# Autodesk Inventor assembly: lemon shape asse
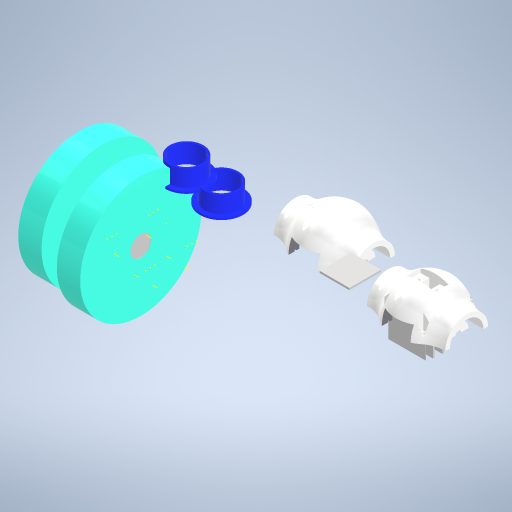
[picture p0: Inventor's stored thumbnail of the model, 512x512]
Saved by Autodesk Inventor 2023 (Build 270158000, 158)
## iProperties
Created: 2022-11-14
Part Number: lemon shape asse
Document SubType Name: Assembly
Designer: RM206user
Author: RM206user
## Documents named in this file (10)
- C:\Users\RM206user\Desktop\cansat\tanekonsat2022_runback\machinary\parts\tire\lemon shape asse.iam
- C:\Users\RM206user\Desktop\cansat\tanekonsat2022_runback\machinary\parts\tire\130 25 lemon tire.iam
- C:\Users\RM206user\Desktop\cansat\tanekonsat2022_runback\machinary\parts\bush.ipt
- C:\Users\RM206user\Desktop\cansat\tanekonsat2022_runback\machinary\body\body back\back moter middle tire ver\back moter middle tire lemon shape.ipt
- C:\Users\RM206user\Desktop\cansat\tanekonsat2022_runback\machinary\body\body front\front moter middle basic\body front moter middle lemon shape.ipt
- C:\Users\RM206user\Desktop\cansat\tanekonsat2022_runback\machinary\body\body back\back for main connection\body back for main 3.ipt
- C:\Users\RM206user\Desktop\cansat\tanekonsat2022_runback\machinary\parts\GNSS1.ipt
- C:\Users\RM206user\Desktop\cansat\tanekonsat2022_runback\machinary\parts\almi1.ipt
- C:\Users\RM206user\Desktop\cansat\tanekonsat2022_runback\machinary\parts\almi2.ipt
- C:\Users\RM206user\Desktop\cansat\tanekonsat2022_runback\machinary\parts\mein1.ipt
## Components (11 placed, 9 different names)
1. 130 25 lemon tire:1 [sub-assembly]
2. 130 25 lemon tire:2 [sub-assembly]
3. bush:1
4. bush:2
5. body moter middle:1 — メイト:1, メイト:2
6. base front:1 — メイト:3, メイト:4, メイト:5, メイト:6, メイト:7, メイト:8, メイト:9
7. body back:1 — メイト:1, メイト:2
8. GNSS1:1
9. almi1:1 — メイト:6, メイト:7
10. almi2:1 — メイト:3, メイト:4, メイト:5
11. mein1:1 — メイト:8, メイト:9
## Relationships (9: Mate 9)
- メイト:1 [Mate]: body moter middle:1 ↔ body back:1
- メイト:2 [Mate]: body moter middle:1 ↔ body back:1
- メイト:3 [Mate]: base front:1 ↔ almi2:1
- メイト:4 [Mate]: base front:1 ↔ almi2:1
- メイト:5 [Mate]: base front:1 ↔ almi2:1
- メイト:6 [Mate]: base front:1 ↔ almi1:1
- メイト:7 [Mate]: base front:1 ↔ almi1:1
- メイト:8 [Mate]: base front:1 ↔ mein1:1
- メイト:9 [Mate]: base front:1 ↔ mein1:1
